# Autodesk Inventor assembly: RaspberryPi-Enclosure
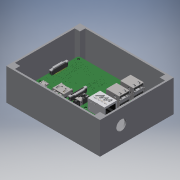
[picture p0: Inventor's stored thumbnail of the model, 180x180]
Saved by Autodesk Inventor 2018 (Build 220112000, 112)
## iProperties
Created: 2018-04-28
Part Number: RaspberryPi-Enclosure
Document SubType Name: Assembly
Designer: bbramman
Author: bbramman
## Documents named in this file (4)
- C:\Users\bbramman\OneDrive\Documents\Trapped Ion Research (Grad)\Electronics\pll-evalboard-synthesizer\Box CAD\RaspberryPi-Enclosure.iam
- C:\Users\bbramman\OneDrive\Documents\Trapped Ion Research (Grad)\Electronics\pll-evalboard-synthesizer\Box CAD\546-1590BBS-Pi.ipt
- C:\Users\bbramman\OneDrive\Documents\Trapped Ion Research (Grad)\Electronics\pll-evalboard-synthesizer\Box CAD\Power-Reg.iam
- C:\Users\bbramman\OneDrive\Documents\Trapped Ion Research (Grad)\Electronics\pll-evalboard-synthesizer\Box CAD\RPi3_ModelB v1.iam
## Components (3 placed, 3 different names)
1. 546-1590BBS-Pi:1 — Insert:1, Insert:2
2. Power-Reg:1 [sub-assembly] — Insert:1
3. RPi3_ModelB v1:1 [sub-assembly] — Insert:2
## Relationships (2: Insert 2)
- Insert:1 (6.35 mm): 546-1590BBS-Pi:1 ↔ Power-Reg:1
- Insert:2 (-21.3106 mm): 546-1590BBS-Pi:1 ↔ RPi3_ModelB v1:1
